# Autodesk Inventor assembly: robotetz
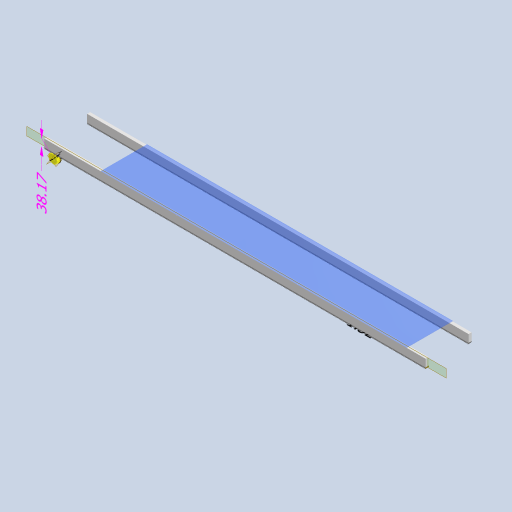
[picture p0: Inventor's stored thumbnail of the model, 512x512]
Saved by Autodesk Inventor 2024.2 (Build 282272000, 272)
## iProperties
Created: 2025-11-16
Part Number: robotetz
Document SubType Name: Assembly
Designer: katya_notebook
Author: katya_notebook
## Documents named in this file (4)
- C:\Users\91125\OneDrive\Рабочий стол\alletz\etz\robotetz.iam
- C:\Users\91125\OneDrive\Рабочий стол\alletz\полигон етз.iam
- C:\Users\91125\OneDrive\Документы\Шестерня.ipt
- C:\Users\91125\OneDrive\Рабочий стол\alletz\муфта.ipt
## Components (3 placed, 3 different names)
1. полигон етз:1 [sub-assembly] — Заподлицо:1, Совмещение:1
2. Шестерня:1 — Заподлицо:1, Совмещение:1, С поворотом:1
3. муфта:1 — С поворотом:1
## Relationships (3: Flush 1, Mate 1, RevoluteJoint 1)
- Заподлицо:1 [Flush]: полигон етз:1 ↔ Шестерня:1
- Совмещение:1 [Mate] (28 mm): полигон етз:1 ↔ Шестерня:1
- С поворотом:1 [RevoluteJoint]: Шестерня:1 ↔ муфта:1
